# Autodesk Inventor assembly: one_servo_test
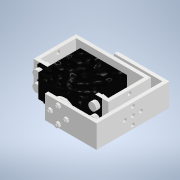
[picture p0: Inventor's stored thumbnail of the model, 180x180]
Saved by Autodesk Inventor 2021.4 (Build 254397000, 397)
## iProperties
Created: 2022-07-24
Part Number: one_servo_test
Document SubType Name: Assembly
Designer: isamu
Author: isamu
## Documents named in this file (3)
- D:\personal_projects\robot\inventor\2021_matlab_compat _v2\tests\one_servo_test.iam
- D:\personal_projects\robot\inventor\2021_matlab_compat _v2\servo_rot_frame\mg996r_rot_frame.iam
- D:\personal_projects\robot\inventor\2021_matlab_compat _v2\motor_with_frames\mg996r_base_motor_with_axis.iam
## Components (2 placed, 2 different names)
1. mg996r_base_motor_with_axis:1 [sub-assembly] — Rotational:1
2. mg996r_rot_frame:1 [sub-assembly] — Rotational:1
## Relationships (1: RevoluteJoint 1)
- Rotational:1 [RevoluteJoint]: mg996r_base_motor_with_axis:1 ↔ mg996r_rot_frame:1
